# Autodesk Inventor assembly: X Axis Motor End_MIR
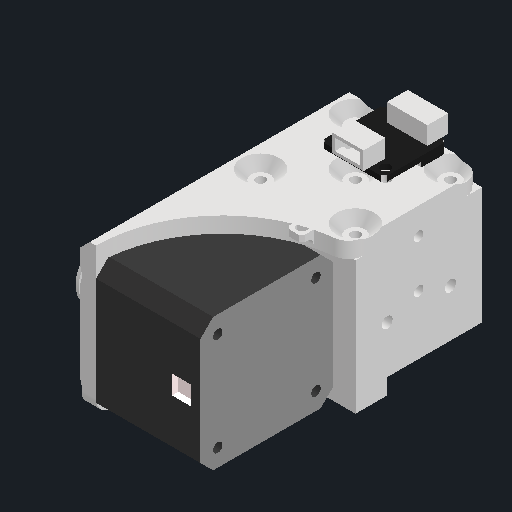
[picture p0: Inventor's stored thumbnail of the model, 512x512]
Saved by Autodesk Inventor 2026 (Build 300175000, 175)
## iProperties
Created: 2025-02-02
Part Number: X Axis Motor End_MIR
Document SubType Name: Assembly
Designer: jerem
Author: jerem
## Documents named in this file (6)
- C:\Users\jerem\Documents\GitHub\Perovskite-Automated-Synthesis-System\CAD\Gantry\X Axis\X Axis Motor End_MIR.iam
- C:\Users\jerem\Documents\GitHub\Perovskite-Automated-Synthesis-System\CAD\Gantry\X Axis\X Axis Rail End.ipt
- C:\Users\jerem\Documents\GitHub\Perovskite-Automated-Synthesis-System\CAD\Non 3D Printed Parts\Motors and Servos\NEMA17 Stepper Motor.ipt
- C:\Users\jerem\Documents\GitHub\Perovskite-Automated-Synthesis-System\CAD\Non 3D Printed Parts\Idler.ipt
- C:\Users\jerem\Documents\GitHub\Perovskite-Automated-Synthesis-System\CAD\Gantry\X Axis\Tensioner End Bracket_MIR1.ipt
- C:\Users\jerem\Documents\GitHub\Perovskite-Automated-Synthesis-System\CAD\Non 3D Printed Parts\Limit Switch.ipt
## Components (5 placed, 5 different names)
1. X Axis Rail End:1 — Mate:5, Mate:7, Mate:8
2. NEMA17 Stepper Motor:1 — Mate:3, Mate:6, Mate:9
3. Idler:1 — Mate:9
4. Tensioner End Bracket_MIR:1 — Mate:1, Mate:2, Mate:3, Mate:4, Mate:5, Mate:6, Mate:7, Mate:8
5. Limit Switch:1 — Mate:1, Mate:2, Mate:4
## Relationships (9: Mate 9)
- Mate:1: Tensioner End Bracket_MIR:1 ↔ Limit Switch:1
- Mate:2: Tensioner End Bracket_MIR:1 ↔ Limit Switch:1
- Mate:3: NEMA17 Stepper Motor:1 ↔ Tensioner End Bracket_MIR:1
- Mate:4: Tensioner End Bracket_MIR:1 ↔ Limit Switch:1
- Mate:5: X Axis Rail End:1 ↔ Tensioner End Bracket_MIR:1
- Mate:6: NEMA17 Stepper Motor:1 ↔ Tensioner End Bracket_MIR:1
- Mate:7: X Axis Rail End:1 ↔ Tensioner End Bracket_MIR:1
- Mate:8: X Axis Rail End:1 ↔ Tensioner End Bracket_MIR:1
- Mate:9: NEMA17 Stepper Motor:1 ↔ Idler:1
